# Autodesk Inventor assembly: Baugruppe1
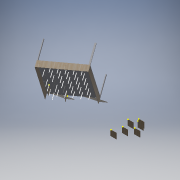
[picture p0: Inventor's stored thumbnail of the model, 180x180]
Saved by Autodesk Inventor 2019 (Build 230136000, 136)
## iProperties
Created: 2021-09-26
Part Number: Baugruppe1
Material: Generisch
Document SubType Name: Assembly
Designer: mritt
Author: mritt
## Documents named in this file (7)
- D:\Studium\Universität Stuttgart\Sonstige Tätigkeiten\Tätigkeit_studentische_Hilfskraft_Informatik\Hiwi-Projekt\CAD-Dateien\Arena\Arena Maze\Baugruppe1.iam
- D:\Studium\Universität Stuttgart\Sonstige Tätigkeiten\Tätigkeit_studentische_Hilfskraft_Informatik\Hiwi-Projekt\CAD-Dateien\Arena\Arena Maze\Bauteil1.ipt
- D:\Studium\Universität Stuttgart\Sonstige Tätigkeiten\Tätigkeit_studentische_Hilfskraft_Informatik\Hiwi-Projekt\CAD-Dateien\Arena\Arena Maze\Bauteil2.ipt
- D:\Studium\Universität Stuttgart\Sonstige Tätigkeiten\Tätigkeit_studentische_Hilfskraft_Informatik\Hiwi-Projekt\CAD-Dateien\Arena\Arena Maze\Bauteil3.ipt
- D:\Studium\Universität Stuttgart\Sonstige Tätigkeiten\Tätigkeit_studentische_Hilfskraft_Informatik\Hiwi-Projekt\CAD-Dateien\Arena\Arena Maze\Wand.ipt
- D:\Studium\Universität Stuttgart\Sonstige Tätigkeiten\Tätigkeit_studentische_Hilfskraft_Informatik\Hiwi-Projekt\CAD-Dateien\Arena\Arena Maze\Füße.ipt
- D:\Studium\Universität Stuttgart\Sonstige Tätigkeiten\Tätigkeit_studentische_Hilfskraft_Informatik\Hiwi-Projekt\CAD-Dateien\Arena\Arena Maze\Rampe.ipt
## Components (54 placed, 6 different names)
1. Bauteil1:1 — Passend:3, Passend:4, Passend:5, Passend:6, Passend:7, Passend:8, Passend:9, Passend:10, Passend:11, Passend:13, Passend:14, Passend:17, Passend:18, Passend:19, Passend:20, Passend:21, Passend:22, Passend:23, Passend:24, Passend:25, Passend:26, Passend:27, Passend:28, Passend:29, Passend:30, Passend:31, Passend:32, Passend:33, Passend:34, Passend:35, Passend:36, Passend:37, Passend:38, Passend:39, Passend:40, Passend:41, Passend:42, Passend:43, Passend:44, Passend:45, Passend:46, Passend:50, Passend:52, Passend:53, Fluchtend:2, Passend:54, Fluchtend:3, Fluchtend:5, Fluchtend:6, Fluchtend:8, Passend:55, Fluchtend:9, Fluchtend:10, Fluchtend:11, Passend:56, Passend:57, Fluchtend:12, Fluchtend:13, Fluchtend:14, Fluchtend:15, Passend:58, Passend:59, Fluchtend:16, Passend:60
2. Bauteil2:1 — Passend:5, Passend:44
3. Bauteil2:2 — Passend:14, Fluchtend:1
4. Bauteil2:3
5. Bauteil2:4 — Passend:7, Passend:49, Passend:51
6. Bauteil2:5 — Passend:8
7. Bauteil2:6 — Passend:10
8. Bauteil2:7 — Passend:11
9. Bauteil2:8 — Passend:6
10. Bauteil2:9 — Passend:13, Fluchtend:1
11. Bauteil2:11 — Passend:9
12. Bauteil2:12 — Passend:3, Passend:4
13. Bauteil2:13 — Passend:17
14. Bauteil2:14 — Passend:31
15. Bauteil2:15 — Passend:18
16. Bauteil2:16 — Passend:19
17. Bauteil2:17 — Passend:20
18. Bauteil2:18 — Passend:21
19. Bauteil2:19 — Passend:22
20. Bauteil2:20 — Passend:23
21. Bauteil2:21 — Passend:24
22. Bauteil2:22 — Passend:25
23. Bauteil2:23 — Passend:27
24. Bauteil2:24 — Passend:26
25. Bauteil2:25 — Passend:30
26. Bauteil2:26 — Passend:29
27. Bauteil2:27 — Passend:28
28. Bauteil2:28 — Passend:34
29. Bauteil2:33 — Passend:39, Passend:42, Passend:47, Passend:48
30. Bauteil2:34 — Passend:38, Passend:45
31. Bauteil2:35 — Passend:32, Passend:46
32. Bauteil2:36 — Passend:37
33. Bauteil2:37 — Passend:36
34. Bauteil2:38 — Passend:35
35. Bauteil2:39 — Passend:40, Passend:43
36. Bauteil2:40 — Passend:33
37. Bauteil2:41 — Passend:41
38. Bauteil3:1 — Passend:47, Passend:48, Passend:52
39. Bauteil3:2
40. Bauteil3:3 — Passend:49, Passend:50, Passend:51
41. Bauteil3:4
42. Bauteil3:5
43. Bauteil3:6
44. Bauteil3:7
45. Bauteil3:8
46. Wand:1 — Passend:53, Fluchtend:2, Fluchtend:4
47. Wand:2 — Fluchtend:5, Fluchtend:6, Fluchtend:7
48. Wand:3 — Passend:54, Fluchtend:3, Fluchtend:4, Fluchtend:7
49. Füße:1 — Fluchtend:14, Fluchtend:15, Passend:58
50. Füße:2 — Passend:57, Fluchtend:12, Fluchtend:13
51. Füße:3 — Fluchtend:10, Fluchtend:11, Passend:56
52. Füße:4 — Fluchtend:8, Passend:55, Fluchtend:9, Passend:62
53. Rampe:1 — Passend:59, Fluchtend:16, Passend:61, Passend:62
54. Rampe:2 — Passend:60, Passend:61
## Relationships (73: Mate 57, Flush 16)
- Passend:3 [Mate]: Bauteil1:1 ↔ Bauteil2:12
- Passend:4 [Mate]: Bauteil1:1 ↔ Bauteil2:12
- Passend:5 [Mate]: Bauteil1:1 ↔ Bauteil2:1
- Passend:6 [Mate]: Bauteil1:1 ↔ Bauteil2:8
- Passend:7 [Mate]: Bauteil1:1 ↔ Bauteil2:4
- Passend:8 [Mate]: Bauteil1:1 ↔ Bauteil2:5
- Passend:9 [Mate]: Bauteil1:1 ↔ Bauteil2:11
- Passend:10 [Mate]: Bauteil1:1 ↔ Bauteil2:6
- Passend:11 [Mate]: Bauteil1:1 ↔ Bauteil2:7
- Passend:13 [Mate]: Bauteil1:1 ↔ Bauteil2:9
- Passend:14 [Mate]: Bauteil1:1 ↔ Bauteil2:2
- Fluchtend:1 [Flush]: Bauteil2:2 ↔ Bauteil2:9
- Passend:17 [Mate]: Bauteil1:1 ↔ Bauteil2:13
- Passend:18 [Mate]: Bauteil1:1 ↔ Bauteil2:15
- Passend:19 [Mate]: Bauteil1:1 ↔ Bauteil2:16
- Passend:20 [Mate]: Bauteil1:1 ↔ Bauteil2:17
- Passend:21 [Mate]: Bauteil1:1 ↔ Bauteil2:18
- Passend:22 [Mate]: Bauteil1:1 ↔ Bauteil2:19
- Passend:23 [Mate]: Bauteil1:1 ↔ Bauteil2:20
- Passend:24 [Mate]: Bauteil1:1 ↔ Bauteil2:21
- Passend:25 [Mate]: Bauteil1:1 ↔ Bauteil2:22
- Passend:26 [Mate]: Bauteil1:1 ↔ Bauteil2:24
- Passend:27 [Mate]: Bauteil1:1 ↔ Bauteil2:23
- Passend:28 [Mate]: Bauteil1:1 ↔ Bauteil2:27
- Passend:29 [Mate]: Bauteil1:1 ↔ Bauteil2:26
- Passend:30 [Mate]: Bauteil1:1 ↔ Bauteil2:25
- Passend:31 [Mate]: Bauteil1:1 ↔ Bauteil2:14
- Passend:32 [Mate]: Bauteil1:1 ↔ Bauteil2:35
- Passend:33 [Mate]: Bauteil1:1 ↔ Bauteil2:40
- Passend:34 [Mate]: Bauteil1:1 ↔ Bauteil2:28
- Passend:35 [Mate]: Bauteil1:1 ↔ Bauteil2:38
- Passend:36 [Mate]: Bauteil1:1 ↔ Bauteil2:37
- Passend:37 [Mate]: Bauteil1:1 ↔ Bauteil2:36
- Passend:38 [Mate]: Bauteil1:1 ↔ Bauteil2:34
- Passend:39 [Mate]: Bauteil1:1 ↔ Bauteil2:33
- Passend:40 [Mate]: Bauteil1:1 ↔ Bauteil2:39
- Passend:41 [Mate]: Bauteil1:1 ↔ Bauteil2:41
- Passend:42 [Mate]: Bauteil1:1 ↔ Bauteil2:33
- Passend:43 [Mate]: Bauteil1:1 ↔ Bauteil2:39
- Passend:44 [Mate]: Bauteil1:1 ↔ Bauteil2:1
- Passend:45 [Mate]: Bauteil1:1 ↔ Bauteil2:34
- Passend:46 [Mate]: Bauteil1:1 ↔ Bauteil2:35
- Passend:47 [Mate]: Bauteil2:33 ↔ Bauteil3:1
- Passend:48 [Mate]: Bauteil2:33 ↔ Bauteil3:1
- Passend:49 [Mate]: Bauteil2:4 ↔ Bauteil3:3
- Passend:50 [Mate]: Bauteil1:1 ↔ Bauteil3:3
- Passend:51 [Mate]: Bauteil2:4 ↔ Bauteil3:3
- Passend:52 [Mate]: Bauteil1:1 ↔ Bauteil3:1
- Passend:53 [Mate]: Bauteil1:1 ↔ Wand:1
- Fluchtend:2 [Flush]: Bauteil1:1 ↔ Wand:1
- Passend:54 [Mate]: Bauteil1:1 ↔ Wand:3
- Fluchtend:3 [Flush]: Bauteil1:1 ↔ Wand:3
- Fluchtend:4 [Flush]: Wand:1 ↔ Wand:3
- Fluchtend:5 [Flush]: Bauteil1:1 ↔ Wand:2
- Fluchtend:6 [Flush]: Bauteil1:1 ↔ Wand:2
- Fluchtend:7 [Flush]: Wand:2 ↔ Wand:3
- Fluchtend:8 [Flush]: Bauteil1:1 ↔ Füße:4
- Passend:55 [Mate]: Bauteil1:1 ↔ Füße:4
- Fluchtend:9 [Flush]: Bauteil1:1 ↔ Füße:4
- Fluchtend:10 [Flush]: Bauteil1:1 ↔ Füße:3
- Fluchtend:11 [Flush]: Bauteil1:1 ↔ Füße:3
- Passend:56 [Mate]: Bauteil1:1 ↔ Füße:3
- Passend:57 [Mate]: Bauteil1:1 ↔ Füße:2
- Fluchtend:12 [Flush]: Bauteil1:1 ↔ Füße:2
- Fluchtend:13 [Flush]: Bauteil1:1 ↔ Füße:2
- Fluchtend:14 [Flush]: Bauteil1:1 ↔ Füße:1
- Fluchtend:15 [Flush]: Bauteil1:1 ↔ Füße:1
- Passend:58 [Mate]: Bauteil1:1 ↔ Füße:1
- Passend:59 [Mate]: Bauteil1:1 ↔ Rampe:1
- Fluchtend:16 [Flush] (-300 mm): Bauteil1:1 ↔ Rampe:1
- Passend:60 [Mate]: Bauteil1:1 ↔ Rampe:2
- Passend:61 [Mate]: Rampe:1 ↔ Rampe:2
- Passend:62 [Mate]: Füße:4 ↔ Rampe:1
